# Autodesk Inventor assembly: 知能ロボコン発射台支え
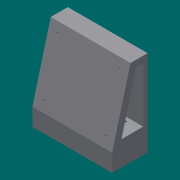
[picture p0: Inventor's stored thumbnail of the model, 180x180]
Saved by Autodesk Inventor 2013 (Build 170138000, 138)
## iProperties
Created: 2014-11-26
Part Number: 知能ロボコン発射台支え
Document SubType Name: Assembly
Designer: horumo136
Author: horumo136
## Documents named in this file (3)
- C:\Users\horumo136\Documents\知能ロボコン発射台支え.iam
- C:\Users\horumo136\Documents\知能ロボコン土台1.1.ipt
- C:\Users\horumo136\Documents\知能ロボコンスペーサ1.1.ipt
## Components (2 placed, 2 different names)
1. 知能ロボコン土台1.1:1 — メイト:1, メイト:2, メイト:3
2. 知能ロボコンスペーサ1.1:1 — メイト:1, メイト:2, メイト:3
## Relationships (3: Mate 3)
- メイト:1 [Mate]: 知能ロボコン土台1.1:1 ↔ 知能ロボコンスペーサ1.1:1
- メイト:2 [Mate]: 知能ロボコン土台1.1:1 ↔ 知能ロボコンスペーサ1.1:1
- メイト:3 [Mate]: 知能ロボコン土台1.1:1 ↔ 知能ロボコンスペーサ1.1:1
